# Autodesk Inventor assembly: Aufhängung
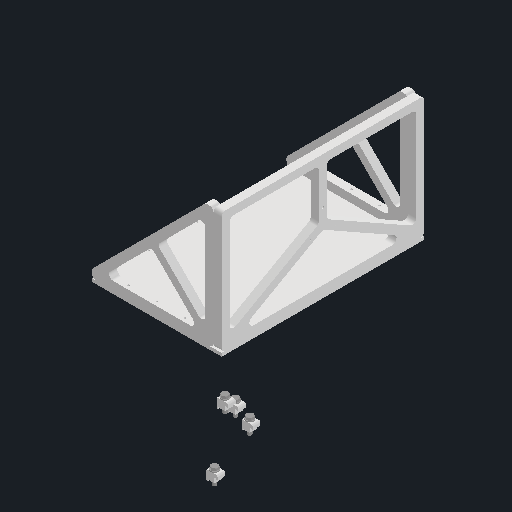
[picture p0: Inventor's stored thumbnail of the model, 512x512]
Saved by Autodesk Inventor 2027 (Build 310192060, 192F)
## iProperties
Created: 2026-07-21
Part Number: Aufhängung
Document SubType Name: Assembly
Designer: kw
Author: kw
## Documents named in this file (5)
- C:\Users\kw\OneDrive\Documents\Uni\Masterthesis\Spezialisierungsmodul\InventorZeichnungen\Koppeltest_Halterung\Aufhängung_RFG.iam
- C:\Users\kw\OneDrive\Documents\Uni\Masterthesis\Spezialisierungsmodul\InventorZeichnungen\Koppeltest_Halterung\Aufhängung_Front_RFG.ipt
- C:\Users\kw\OneDrive\Documents\Uni\Masterthesis\Spezialisierungsmodul\InventorZeichnungen\Koppeltest_Halterung\Aufhängung_Seitenteil.ipt
- C:\Users\kw\OneDrive\Documents\Uni\Masterthesis\Spezialisierungsmodul\InventorZeichnungen\Koppeltest_Halterung\Halterung_Teflonplatte.ipt
- C:\Users\kw\OneDrive\Documents\Uni\Masterthesis\Spezialisierungsmodul\InventorZeichnungen\Koppeltest_Halterung\Pratze_ISO-K160.ipt
## Components (8 placed, 4 different names)
1. Aufhängung_Front_RFG:1 — Mate:3, Flush:5, Flush:6
2. Aufhängung_Seitenteil:1 — Mate:1, Flush:1, Flush:2
3. Halterung_Teflonplatte:1 — Mate:1, Flush:1, Flush:2, Mate:2, Flush:3, Flush:4, Mate:3, Flush:5, Flush:6
4. Aufhängung_Seitenteil:2 — Mate:2, Flush:3, Flush:4
5. Pratze_ISO-K160:1
6. Pratze_ISO-K160:2
7. Pratze_ISO-K160:3
8. Pratze_ISO-K160:4
## Relationships (9: Flush 6, Mate 3)
- Mate:1: Aufhängung_Seitenteil:1 ↔ Halterung_Teflonplatte:1
- Flush:1: Aufhängung_Seitenteil:1 ↔ Halterung_Teflonplatte:1
- Flush:2 (20 mm): Aufhängung_Seitenteil:1 ↔ Halterung_Teflonplatte:1
- Mate:2: Halterung_Teflonplatte:1 ↔ Aufhängung_Seitenteil:2
- Flush:3: Halterung_Teflonplatte:1 ↔ Aufhängung_Seitenteil:2
- Flush:4 (20 mm): Halterung_Teflonplatte:1 ↔ Aufhängung_Seitenteil:2
- Mate:3: Aufhängung_Front_RFG:1 ↔ Halterung_Teflonplatte:1
- Flush:5: Aufhängung_Front_RFG:1 ↔ Halterung_Teflonplatte:1
- Flush:6: Aufhängung_Front_RFG:1 ↔ Halterung_Teflonplatte:1
